# Autodesk Inventor assembly: Sierra
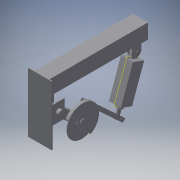
[picture p0: Inventor's stored thumbnail of the model, 180x180]
Saved by Autodesk Inventor 2018 (Build 220112000, 112)
## iProperties
Created: 2021-07-10
Part Number: Sierra
Material: Genérico
Document SubType Name: Assembly
Designer: GABRIEL
Author: GABRIEL
## Documents named in this file (13)
- C:\Users\GABRIEL\Documents\Gabriel\UNAL\SEMESTRE XI\Automatización de PM\Proyecto\Maquina de boca de pescado\Sierra.iam
- C:\Users\GABRIEL\Documents\Gabriel\UNAL\SEMESTRE XI\Automatización de PM\Proyecto\Maquina de boca de pescado\Base sierra.ipt
- C:\Users\GABRIEL\Documents\Gabriel\UNAL\SEMESTRE XI\Automatización de PM\Proyecto\Maquina de boca de pescado\sierra corte.ipt
- C:\Users\GABRIEL\Documents\Gabriel\UNAL\SEMESTRE XI\Automatización de PM\Proyecto\Maquina de boca de pescado\protector.ipt
- C:\Users\GABRIEL\Documents\Gabriel\UNAL\SEMESTRE XI\Automatización de PM\Proyecto\Maquina de boca de pescado\pasador.ipt
- C:\Users\GABRIEL\Documents\Gabriel\UNAL\SEMESTRE XI\Automatización de PM\Proyecto\Maquina de boca de pescado\soporte.ipt
- C:\Users\GABRIEL\Documents\Gabriel\UNAL\SEMESTRE XI\Automatización de PM\Proyecto\Maquina de boca de pescado\Sop vertical.ipt
- C:\Users\GABRIEL\Documents\Gabriel\UNAL\SEMESTRE XI\Automatización de PM\Proyecto\Maquina de boca de pescado\codo.ipt
- C:\Users\GABRIEL\Documents\Gabriel\UNAL\SEMESTRE XI\Automatización de PM\Proyecto\Maquina de boca de pescado\brazo.ipt
- C:\Users\GABRIEL\Documents\Gabriel\UNAL\SEMESTRE XI\Automatización de PM\Proyecto\Maquina de boca de pescado\pasadores brazo.ipt
- C:\Users\GABRIEL\Documents\Gabriel\UNAL\SEMESTRE XI\Automatización de PM\Proyecto\Maquina de boca de pescado\cilindro sierra.ipt
- C:\Users\GABRIEL\Documents\Gabriel\UNAL\SEMESTRE XI\Automatización de PM\Proyecto\Maquina de boca de pescado\cil_sierra.ipt
- C:\Users\GABRIEL\Documents\Gabriel\UNAL\SEMESTRE XI\Automatización de PM\Proyecto\Maquina de boca de pescado\soporte vertical.ipt
## Components (18 placed, 12 different names)
1. Base sierra:1 — Coincidencia:4, Coincidencia:5, Coincidencia:6, Nivelación:4, Nivelación:5, Coincidencia:9, Nivelación:7, Nivelación:8
2. sierra corte:1 — Coincidencia:2, Nivelación:1
3. protector:1 — Coincidencia:1, Coincidencia:3, Nivelación:2, Coincidencia:13, Ángulo:1, Coincidencia:14, Ángulo:2, Coincidencia:15, Coincidencia:20, Tangente:1
4. pasador:1 — Coincidencia:2, Nivelación:1, Coincidencia:3, Nivelación:2, Coincidencia:12
5. soporte:1 — Coincidencia:4, Coincidencia:5, Coincidencia:7, Nivelación:3, Nivelación:4, Nivelación:5, Nivelación:6, Coincidencia:11
6. soporte:2 — Coincidencia:6, Coincidencia:7, Nivelación:3, Coincidencia:8
7. codo:1 — Coincidencia:10, Coincidencia:11, Coincidencia:12, Coincidencia:13, Ángulo:1
8. pasador:2 — Coincidencia:8, Nivelación:6, Coincidencia:10
9. Sop vertical:1 — Coincidencia:9, Nivelación:7, Nivelación:8, Coincidencia:23, Nivelación:12, Coincidencia:24, Nivelación:13
10. brazo:1 — Coincidencia:18, Coincidencia:19, Coincidencia:20, Coincidencia:22, Nivelación:11
11. pasadores brazo:1 — Coincidencia:14, Ángulo:2, Coincidencia:15, Coincidencia:18, Nivelación:9
12. pasadores brazo:2 — Coincidencia:19, Tangente:1, Nivelación:9
13. pasadores brazo:3 — Coincidencia:22, Nivelación:11, Coincidencia:28
14. cilindro sierra:1 — Coincidencia:21, Nivelación:10, Ángulo:3, Coincidencia:26, Coincidencia:27
15. cil_sierra:1 — Coincidencia:21, Nivelación:10, Ángulo:3, Coincidencia:28
16. soporte vertical:1 — Coincidencia:23, Nivelación:12, Nivelación:13, Nivelación:14, Coincidencia:27, Nivelación:17
17. soporte vertical:2 — Coincidencia:24, Nivelación:14, Coincidencia:25, Nivelación:16, Nivelación:17
18. pasadores brazo:4 — Coincidencia:25, Nivelación:16, Coincidencia:26
## Relationships (46: Mate 26, Flush 16, Angle 3, Tangent 1)
- Coincidencia:1 [Mate]: protector:1
- Coincidencia:2 [Mate]: sierra corte:1 ↔ pasador:1
- Nivelación:1 [Flush] (5 mm): sierra corte:1 ↔ pasador:1
- Coincidencia:3 [Mate]: protector:1 ↔ pasador:1
- Nivelación:2 [Flush] (2 mm): protector:1 ↔ pasador:1
- Coincidencia:4 [Mate]: Base sierra:1 ↔ soporte:1
- Coincidencia:5 [Mate]: Base sierra:1 ↔ soporte:1
- Coincidencia:6 [Mate]: Base sierra:1 ↔ soporte:2
- Coincidencia:7 [Mate] (30 mm): soporte:1 ↔ soporte:2
- Nivelación:3 [Flush]: soporte:1 ↔ soporte:2
- Nivelación:4 [Flush] (20 mm): Base sierra:1 ↔ soporte:1
- Nivelación:5 [Flush] (100 mm): Base sierra:1 ↔ soporte:1
- Coincidencia:8 [Mate]: soporte:2 ↔ pasador:2
- Nivelación:6 [Flush]: soporte:1 ↔ pasador:2
- Coincidencia:9 [Mate]: Base sierra:1 ↔ Sop vertical:1
- Nivelación:7 [Flush] (10 mm): Base sierra:1 ↔ Sop vertical:1
- Nivelación:8 [Flush] (10 mm): Base sierra:1 ↔ Sop vertical:1
- Coincidencia:10 [Mate]: codo:1 ↔ pasador:2
- Coincidencia:11 [Mate]: soporte:1 ↔ codo:1
- Coincidencia:12 [Mate]: pasador:1 ↔ codo:1
- Coincidencia:13 [Mate]: protector:1 ↔ codo:1
- Ángulo:1 [Angle] (10 deg): protector:1 ↔ codo:1
- Coincidencia:14 [Mate]: protector:1 ↔ pasadores brazo:1
- Ángulo:2 [Angle] (0 deg): protector:1 ↔ pasadores brazo:1
- Coincidencia:15 [Mate]: protector:1 ↔ pasadores brazo:1
- Coincidencia:18 [Mate]: brazo:1 ↔ pasadores brazo:1
- Coincidencia:19 [Mate]: brazo:1 ↔ pasadores brazo:2
- Coincidencia:20 [Mate]: protector:1 ↔ brazo:1
- Tangente:1 (-4 mm): protector:1 ↔ pasadores brazo:2
- Nivelación:9 [Flush]: pasadores brazo:1 ↔ pasadores brazo:2
- Coincidencia:21 [Mate]: cilindro sierra:1 ↔ cil_sierra:1
- Nivelación:10 [Flush]: cilindro sierra:1 ↔ cil_sierra:1
- Coincidencia:22 [Mate]: brazo:1 ↔ pasadores brazo:3
- Nivelación:11 [Flush] (-1 mm): brazo:1 ↔ pasadores brazo:3
- Ángulo:3 [Angle] (0 deg): cilindro sierra:1 ↔ cil_sierra:1
- Coincidencia:23 [Mate]: Sop vertical:1 ↔ soporte vertical:1
- Nivelación:12 [Flush] (20 mm): Sop vertical:1 ↔ soporte vertical:1
- Coincidencia:24 [Mate]: Sop vertical:1 ↔ soporte vertical:2
- Nivelación:13 [Flush] (10 mm): Sop vertical:1 ↔ soporte vertical:1
- Nivelación:14 [Flush] (15 mm): soporte vertical:1 ↔ soporte vertical:2
- Coincidencia:25 [Mate]: soporte vertical:2 ↔ pasadores brazo:4
- Nivelación:16 [Flush] (-1 mm): soporte vertical:2 ↔ pasadores brazo:4
- Coincidencia:26 [Mate]: cilindro sierra:1 ↔ pasadores brazo:4
- Coincidencia:27 [Mate]: cilindro sierra:1 ↔ soporte vertical:1
- Coincidencia:28 [Mate]: pasadores brazo:3 ↔ cil_sierra:1
- Nivelación:17 [Flush]: soporte vertical:1 ↔ soporte vertical:2
